# Autodesk Inventor assembly: OttosAssembly
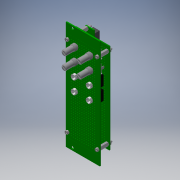
[picture p0: Inventor's stored thumbnail of the model, 180x180]
Saved by Autodesk Inventor 2016 (Build 200138000, 138)
## iProperties
Created: 2018-01-08
Part Number: OttosAssembly
Document SubType Name: Assembly
Designer: suku
Author: suku
## Documents named in this file (10)
- I:\SukuWc\Eurorack\DIY\pcb\Assembly\OttosAssembly.iam
- I:\SukuWc\Eurorack\DIY\pcb\Assembly\Powerbrick.ipt
- I:\SukuWc\Eurorack\DIY\pcb\Assembly\Stripboard-480.ipt
- I:\SukuWc\Eurorack\DIY\pcb\Assembly\cut.ipt
- I:\SukuWc\Eurorack\DIY\pcb\Assembly\rail.ipt
- I:\SukuWc\Eurorack\DIY\pcb\Assembly\P0915N-EC15BR10K.ipt
- I:\SukuWc\Eurorack\DIY\pcb\Assembly\M2x12 HEX SPACER.ipt
- C:\Users\suku\Documents\Inventor\Content Center Files\R2016\en-US\ANSI B18.3.1M(1)\ANSI B18.3.1M - M2x0.4 x 8(2).ipt
- C:\Users\suku\Documents\Inventor\Content Center Files\R2016\en-US\BS 3692(1)\BS 3692 - M2(1).ipt
- I:\SukuWc\Eurorack\DIY\pcb\Assembly\KNOBICONN_TRS.ipt
## Components (27 placed, 9 different names)
1. Powerbrick:1 — Mate:1, Mate:2, Mate:30, Mate:32, Mate:41, Mate:55, Mate:56
2. Stripboard-480:1 — Mate:1, Mate:2, Mate:3, Mate:4, Mate:19, Mate:20, Mate:21, Mate:22, Mate:24, Mate:25, Mate:27, Mate:28, Mate:42, Mate:43, Mate:44, Mate:45, Mate:46, Mate:47, Mate:48, Mate:49, Mate:50, Mate:63, Mate:64, Mate:65, Mate:66
3. cut:1 — Mate:3, Mate:4, Mate:23, Mate:29, Mate:31, Mate:33, Mate:34, Mate:35, Mate:36, Mate:37, Mate:38, Mate:39, Mate:40, Mate:57, Mate:58, Mate:67, Mate:68, Mate:69, Mate:70
4. rail:1 — Mate:19, Mate:21, Flush:1
5. rail:2 — Mate:20, Mate:22, Flush:1
6. P0915N-EC15BR10K:1 — Flush:3, Mate:28
7. P0915N-EC15BR10K:2 — Flush:4, Mate:27
8. P0915N-EC15BR10K:3 — Mate:25, Flush:2, Flush:4
9. P0915N-EC15BR10K:4 — Mate:23, Mate:24, Flush:2, Flush:3
10. M2x12 HEX SPACER:1 — Mate:29, Mate:35
11. M2x12 HEX SPACER:2 — Mate:31, Mate:36
12. M2x12 HEX SPACER:3 — Mate:32, Mate:40, Mate:53
13. M2x12 HEX SPACER:4 — Mate:30, Mate:39, Mate:41, Mate:54
14. M2x12 HEX SPACER:5 — Mate:34, Mate:37, Mate:51
15. M2x12 HEX SPACER:6 — Mate:33, Mate:38, Mate:42, Mate:52
16. Broached Socket Head Cap Screw - Metric M2x0.4 x 8:1 — Mate:43, Mate:47
17. Broached Socket Head Cap Screw - Metric M2x0.4 x 8:2 — Mate:44, Mate:49
18. Broached Socket Head Cap Screw - Metric M2x0.4 x 8:3 — Mate:46, Mate:50
19. Broached Socket Head Cap Screw - Metric M2x0.4 x 8:4 — Mate:45, Mate:48
20. BS 3692 - Metric M2:1 — Mate:51, Mate:58
21. BS 3692 - Metric M2:2 — Mate:53, Mate:55
22. BS 3692 - Metric M2:3 — Mate:52, Mate:57
23. BS 3692 - Metric M2:4 — Mate:54, Mate:56
24. KNOBICONN_TRS:1 — Mate:63, Flush:5, Mate:68
25. KNOBICONN_TRS:2 — Mate:65, Flush:5, Flush:6, Mate:67
26. KNOBICONN_TRS:3 — Mate:64, Flush:7, Mate:69
27. KNOBICONN_TRS:4 — Mate:66, Flush:6, Flush:7, Mate:70
## Relationships (58: Mate 51, Flush 7)
- Mate:1: Powerbrick:1 ↔ Stripboard-480:1
- Mate:2: Powerbrick:1 ↔ Stripboard-480:1
- Mate:3: Stripboard-480:1 ↔ cut:1
- Mate:4: Stripboard-480:1 ↔ cut:1
- Mate:19: Stripboard-480:1 ↔ rail:1
- Mate:20: Stripboard-480:1 ↔ rail:2
- Mate:21 (0.1 mm): Stripboard-480:1 ↔ rail:1
- Mate:22 (0.1 mm): Stripboard-480:1 ↔ rail:2
- Flush:1: rail:1 ↔ rail:2
- Mate:23: cut:1 ↔ P0915N-EC15BR10K:4
- Mate:24: Stripboard-480:1 ↔ P0915N-EC15BR10K:4
- Mate:25: Stripboard-480:1 ↔ P0915N-EC15BR10K:3
- Flush:2: P0915N-EC15BR10K:3 ↔ P0915N-EC15BR10K:4
- Flush:3: P0915N-EC15BR10K:1 ↔ P0915N-EC15BR10K:4
- Flush:4: P0915N-EC15BR10K:2 ↔ P0915N-EC15BR10K:3
- Mate:27: Stripboard-480:1 ↔ P0915N-EC15BR10K:2
- Mate:28: Stripboard-480:1 ↔ P0915N-EC15BR10K:1
- Mate:29: cut:1 ↔ M2x12 HEX SPACER:1
- Mate:30: Powerbrick:1 ↔ M2x12 HEX SPACER:4
- Mate:31: cut:1 ↔ M2x12 HEX SPACER:2
- Mate:32: Powerbrick:1 ↔ M2x12 HEX SPACER:3
- Mate:33: cut:1 ↔ M2x12 HEX SPACER:6
- Mate:34: cut:1 ↔ M2x12 HEX SPACER:5
- Mate:35: cut:1 ↔ M2x12 HEX SPACER:1
- Mate:36: cut:1 ↔ M2x12 HEX SPACER:2
- Mate:37: cut:1 ↔ M2x12 HEX SPACER:5
- Mate:38: cut:1 ↔ M2x12 HEX SPACER:6
- Mate:39: cut:1 ↔ M2x12 HEX SPACER:4
- Mate:40: cut:1 ↔ M2x12 HEX SPACER:3
- Mate:41: Powerbrick:1 ↔ M2x12 HEX SPACER:4
- Mate:42: Stripboard-480:1 ↔ M2x12 HEX SPACER:6
- Mate:43: Stripboard-480:1 ↔ Broached Socket Head Cap Screw - Metric M2x0.4 x 8:1
- Mate:44: Stripboard-480:1 ↔ Broached Socket Head Cap Screw - Metric M2x0.4 x 8:2
- Mate:45: Stripboard-480:1 ↔ Broached Socket Head Cap Screw - Metric M2x0.4 x 8:4
- Mate:46: Stripboard-480:1 ↔ Broached Socket Head Cap Screw - Metric M2x0.4 x 8:3
- Mate:47: Stripboard-480:1 ↔ Broached Socket Head Cap Screw - Metric M2x0.4 x 8:1
- Mate:48: Stripboard-480:1 ↔ Broached Socket Head Cap Screw - Metric M2x0.4 x 8:4
- Mate:49: Stripboard-480:1 ↔ Broached Socket Head Cap Screw - Metric M2x0.4 x 8:2
- Mate:50: Stripboard-480:1 ↔ Broached Socket Head Cap Screw - Metric M2x0.4 x 8:3
- Mate:51: M2x12 HEX SPACER:5 ↔ BS 3692 - Metric M2:1
- Mate:52: M2x12 HEX SPACER:6 ↔ BS 3692 - Metric M2:3
- Mate:53: M2x12 HEX SPACER:3 ↔ BS 3692 - Metric M2:2
- Mate:54: M2x12 HEX SPACER:4 ↔ BS 3692 - Metric M2:4
- Mate:55: Powerbrick:1 ↔ BS 3692 - Metric M2:2
- Mate:56: Powerbrick:1 ↔ BS 3692 - Metric M2:4
- Mate:57: cut:1 ↔ BS 3692 - Metric M2:3
- Mate:58: cut:1 ↔ BS 3692 - Metric M2:1
- Mate:63: Stripboard-480:1 ↔ KNOBICONN_TRS:1
- Mate:64: Stripboard-480:1 ↔ KNOBICONN_TRS:3
- Mate:65: Stripboard-480:1 ↔ KNOBICONN_TRS:2
- Mate:66: Stripboard-480:1 ↔ KNOBICONN_TRS:4
- Flush:5: KNOBICONN_TRS:1 ↔ KNOBICONN_TRS:2
- Flush:6: KNOBICONN_TRS:2 ↔ KNOBICONN_TRS:4
- Flush:7: KNOBICONN_TRS:3 ↔ KNOBICONN_TRS:4
- Mate:67: cut:1 ↔ KNOBICONN_TRS:2
- Mate:68: cut:1 ↔ KNOBICONN_TRS:1
- Mate:69: cut:1 ↔ KNOBICONN_TRS:3
- Mate:70: cut:1 ↔ KNOBICONN_TRS:4
